# Autodesk Inventor assembly: 2024-210-Shootaur-Superstructure
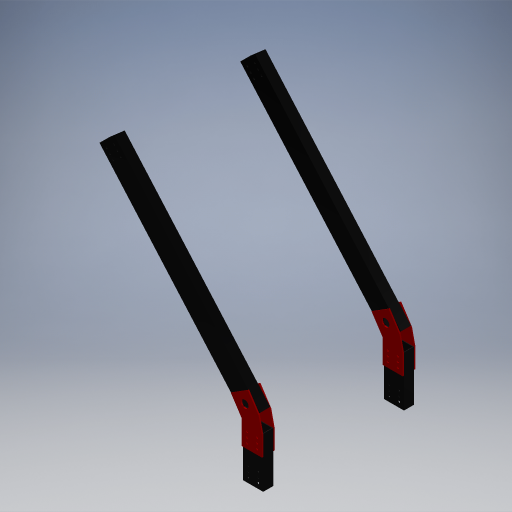
[picture p0: Inventor's stored thumbnail of the model, 512x512]
Saved by Autodesk Inventor 2024.2 (Build 282272000, 272)
## iProperties
Created: 2024-01-21
Part Number: 2024-210-Shootaur-Superstructure
Document SubType Name: Assembly
Designer: rohan
Author: rohan
## Documents named in this file (4)
- C:\Users\rohan\OneDrive - Hillsborough County Public Schools\Robotics\FIRST-Robotics-Competition\Crescendo\Minotaur-Crescendo-Robot\Structure\Superstructure\2024-210-Shootaur-Superstructure.iam
- C:\Users\rohan\OneDrive - Hillsborough County Public Schools\Robotics\FIRST-Robotics-Competition\Crescendo\Minotaur-Crescendo-Robot\Structure\Superstructure\2024-210-001-Angle-Beam.ipt
- C:\Users\rohan\OneDrive - Hillsborough County Public Schools\Robotics\FIRST-Robotics-Competition\Crescendo\Minotaur-Crescendo-Robot\Structure\Superstructure\2024-210-002-Dead-Axle-Gusset.ipt
- C:\Users\rohan\OneDrive - Hillsborough County Public Schools\Robotics\FIRST-Robotics-Competition\Crescendo\Minotaur-Crescendo-Robot\Structure\Superstructure\2024-210-003-Back-Upright.ipt
## Components (8 placed, 3 different names)
1. 2024-210-001-Angle-Beam:1 — Mate:4, Insert:6, Flush:7, Symmetry:1
2. 2024-210-001-Angle-Beam:2 — Mate:3, Insert:5, Flush:7, Symmetry:1, Mate:7
3. 2024-210-002-Dead-Axle-Gusset:1 — Flush:1, Flush:2, Insert:1, Insert:3, Mate:3, Insert:5
4. 2024-210-002-Dead-Axle-Gusset:2 — Flush:1, Flush:2, Insert:1, Flush:5, Mate:1
5. 2024-210-002-Dead-Axle-Gusset:3 — Flush:3, Flush:4, Insert:2, Flush:6, Insert:4, Mate:4, Insert:6
6. 2024-210-002-Dead-Axle-Gusset:4 — Flush:3, Flush:4, Insert:2, Mate:2
7. 2024-210-003-Back-Upright:1 — Flush:5, Mate:1, Insert:3, Flush:8, Mate:5, Mate:6, Flush:9
8. 2024-210-003-Back-Upright:2 — Flush:6, Mate:2, Insert:4, Flush:8, Mate:5, Flush:9
## Relationships (23: Flush 9, Mate 7, Insert 6, Symmetry 1)
- Flush:1: 2024-210-002-Dead-Axle-Gusset:1 ↔ 2024-210-002-Dead-Axle-Gusset:2
- Flush:2: 2024-210-002-Dead-Axle-Gusset:1 ↔ 2024-210-002-Dead-Axle-Gusset:2
- Insert:1 (25.4 mm): 2024-210-002-Dead-Axle-Gusset:1 ↔ 2024-210-002-Dead-Axle-Gusset:2
- Flush:3: 2024-210-002-Dead-Axle-Gusset:3 ↔ 2024-210-002-Dead-Axle-Gusset:4
- Flush:4: 2024-210-002-Dead-Axle-Gusset:3 ↔ 2024-210-002-Dead-Axle-Gusset:4
- Insert:2 (25.4 mm): 2024-210-002-Dead-Axle-Gusset:3 ↔ 2024-210-002-Dead-Axle-Gusset:4
- Flush:5: 2024-210-002-Dead-Axle-Gusset:2 ↔ 2024-210-003-Back-Upright:1
- Mate:1: 2024-210-002-Dead-Axle-Gusset:2 ↔ 2024-210-003-Back-Upright:1
- Insert:3: 2024-210-002-Dead-Axle-Gusset:1 ↔ 2024-210-003-Back-Upright:1
- Flush:6: 2024-210-002-Dead-Axle-Gusset:3 ↔ 2024-210-003-Back-Upright:2
- Mate:2: 2024-210-002-Dead-Axle-Gusset:4 ↔ 2024-210-003-Back-Upright:2
- Insert:4: 2024-210-002-Dead-Axle-Gusset:3 ↔ 2024-210-003-Back-Upright:2
- Mate:3: 2024-210-001-Angle-Beam:2 ↔ 2024-210-002-Dead-Axle-Gusset:1
- Insert:5: 2024-210-001-Angle-Beam:2 ↔ 2024-210-002-Dead-Axle-Gusset:1
- Mate:4: 2024-210-001-Angle-Beam:1 ↔ 2024-210-002-Dead-Axle-Gusset:3
- Insert:6: 2024-210-001-Angle-Beam:1 ↔ 2024-210-002-Dead-Axle-Gusset:3
- Flush:7: 2024-210-001-Angle-Beam:1 ↔ 2024-210-001-Angle-Beam:2
- Flush:8: 2024-210-003-Back-Upright:1 ↔ 2024-210-003-Back-Upright:2
- Mate:5 (330.2 mm): 2024-210-003-Back-Upright:1 ↔ 2024-210-003-Back-Upright:2
- Mate:6: 2024-210-003-Back-Upright:1
- Symmetry:1: 2024-210-001-Angle-Beam:1 ↔ 2024-210-001-Angle-Beam:2
- Mate:7: 2024-210-001-Angle-Beam:2
- Flush:9: 2024-210-003-Back-Upright:1 ↔ 2024-210-003-Back-Upright:2
